# Autodesk Inventor assembly: TOWER PRO MG-995, ANALOG SERVO
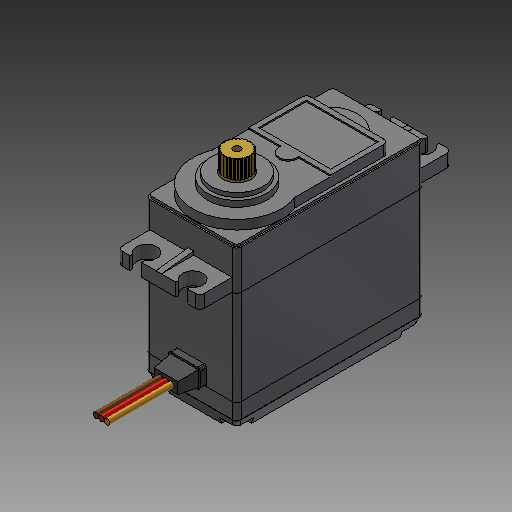
[picture p0: Inventor's stored thumbnail of the model, 512x512]
Saved by Autodesk Inventor 2017 (Build 210142000, 142)
## iProperties
Created: 2014-11-22
Part Number: TOWER PRO MG-995, ANALOG SERVO
Material: Ogólny
Document SubType Name: Assembly
Designer: Speed King
Mass: 31.9788 g
Surface Area: 108.511 cm^2
Volume: 30.6122 cm^3
Density: 1.04464 g/cm^3
Sending System: SolidWorks 2014
Last Author: falcon
Last Saved: 2014-12-08
Author: Speed King
## Documents named in this file (6)
- C:\Users\Speed King\Documents\My Inventor\GrabCAD\Technical Informatics\CAD\model\Tower Pro MG955\TOWER PRO MG-995, ANALOG SERVO.iam
- C:\Users\Speed King\Documents\My Inventor\GrabCAD\Technical Informatics\CAD\model\Tower Pro MG955\TOWER PRO MG-995, ANALOG SERVO, BODY, BOTTOM.ipt
- C:\Users\Speed King\Documents\My Inventor\GrabCAD\Technical Informatics\CAD\model\Tower Pro MG955\TOWER PRO MG-995, ANALOG SERVO, BODY, MIDDLE.ipt
- C:\Users\Speed King\Documents\My Inventor\GrabCAD\Technical Informatics\CAD\model\Tower Pro MG955\TOWER PRO MG-995, ANALOG SERVO, BODY, TOP.ipt
- C:\Users\Speed King\Documents\My Inventor\GrabCAD\Technical Informatics\CAD\model\Tower Pro MG955\TOWER PRO MG-995, ANALOG SERVO, CONNECTOR.ipt
- C:\Users\Speed King\Documents\My Inventor\GrabCAD\Technical Informatics\CAD\model\Tower Pro MG955\TOWER PRO MG-995, ANALOG SERVO, SHAFT.ipt
## Components (5 placed, 5 different names)
1. TOWER PRO MG-995, ANALOG SERVO, BODY, BOTTOM:1 — Zestawiający:2, Równoległy:3, Równoległy:4
2. TOWER PRO MG-995, ANALOG SERVO, BODY, MIDDLE:2 — Równoległy:1, Równoległy:2, Zestawiający:1, Zestawiający:2, Równoległy:3, Równoległy:4, Zestawiający:3, Zestawiający:4, Kąt:1, Zestawiający:9
3. TOWER PRO MG-995, ANALOG SERVO, BODY, TOP:1 — Równoległy:1, Równoległy:2, Zestawiający:1, Zestawiający:5
4. TOWER PRO MG-995, ANALOG SERVO, CONNECTOR:1 — Zestawiający:3, Zestawiający:8, Zestawiający:9
5. TOWER PRO MG-995, ANALOG SERVO, SHAFT:1 — Zestawiający:4, Zestawiający:5, Zestawiający:6, Zestawiający:7, Równoległy:5
## Relationships (15: Mate 9, Flush 5, Angle 1)
- Równoległy:1 [Flush]: TOWER PRO MG-995, ANALOG SERVO, BODY, MIDDLE:2 ↔ TOWER PRO MG-995, ANALOG SERVO, BODY, TOP:1
- Równoległy:2 [Flush]: TOWER PRO MG-995, ANALOG SERVO, BODY, MIDDLE:2 ↔ TOWER PRO MG-995, ANALOG SERVO, BODY, TOP:1
- Zestawiający:1 [Mate]: TOWER PRO MG-995, ANALOG SERVO, BODY, MIDDLE:2 ↔ TOWER PRO MG-995, ANALOG SERVO, BODY, TOP:1
- Zestawiający:2 [Mate]: TOWER PRO MG-995, ANALOG SERVO, BODY, BOTTOM:1 ↔ TOWER PRO MG-995, ANALOG SERVO, BODY, MIDDLE:2
- Równoległy:3 [Flush]: TOWER PRO MG-995, ANALOG SERVO, BODY, BOTTOM:1 ↔ TOWER PRO MG-995, ANALOG SERVO, BODY, MIDDLE:2
- Równoległy:4 [Flush]: TOWER PRO MG-995, ANALOG SERVO, BODY, BOTTOM:1 ↔ TOWER PRO MG-995, ANALOG SERVO, BODY, MIDDLE:2
- Zestawiający:3 [Mate]: TOWER PRO MG-995, ANALOG SERVO, BODY, MIDDLE:2 ↔ TOWER PRO MG-995, ANALOG SERVO, CONNECTOR:1
- Zestawiający:4 [Mate]: TOWER PRO MG-995, ANALOG SERVO, BODY, MIDDLE:2 ↔ TOWER PRO MG-995, ANALOG SERVO, SHAFT:1
- Zestawiający:5 [Mate]: TOWER PRO MG-995, ANALOG SERVO, BODY, TOP:1 ↔ TOWER PRO MG-995, ANALOG SERVO, SHAFT:1
- Zestawiający:6 [Mate]: TOWER PRO MG-995, ANALOG SERVO, SHAFT:1
- Zestawiający:7 [Mate]: TOWER PRO MG-995, ANALOG SERVO, SHAFT:1
- Równoległy:5 [Flush]: TOWER PRO MG-995, ANALOG SERVO, SHAFT:1
- Kąt:1 [Angle] (180 deg): TOWER PRO MG-995, ANALOG SERVO, BODY, MIDDLE:2
- Zestawiający:8 [Mate]: TOWER PRO MG-995, ANALOG SERVO, CONNECTOR:1
- Zestawiający:9 [Mate]: TOWER PRO MG-995, ANALOG SERVO, BODY, MIDDLE:2 ↔ TOWER PRO MG-995, ANALOG SERVO, CONNECTOR:1
